# Autodesk Inventor assembly: cellSTORM_v5_microsocpe_alliedvision
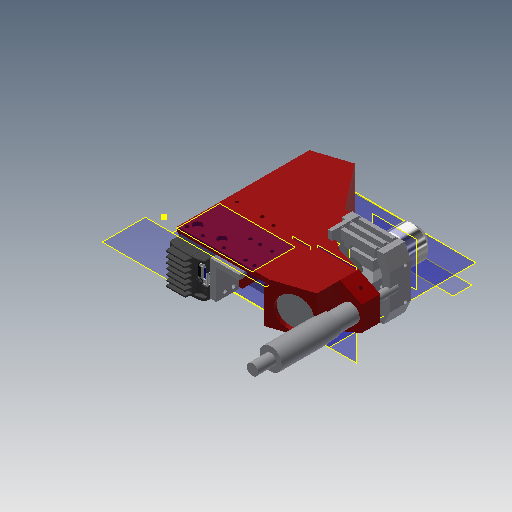
[picture p0: Inventor's stored thumbnail of the model, 512x512]
Saved by Autodesk Inventor 2019.4 (Build 234330000, 330)
## iProperties
Created: 2020-04-25
Part Number: cellSTORM_v5_microsocpe_alliedvision
Document SubType Name: Assembly
Designer: diederichbenedict
Author: diederichbenedict
## Documents named in this file (9)
- C:\Users\diederichbenedict\Dropbox\Dokumente\Promotion\PROJECTS\STORMoChip\GITHUB\CAD\Nanoscopy-on-the-cheap\Workspace\cellSTORM_v5_microsocpe_alliedvision.iam
- C:\Users\diederichbenedict\Dropbox\Dokumente\Promotion\PROJECTS\STORMoChip\GITHUB\CAD\Nanoscopy-on-the-cheap\Workspace\10_Filteslide_25mm.ipt
- C:\Users\diederichbenedict\Dropbox\Dokumente\Promotion\PROJECTS\STORMoChip\GITHUB\CAD\Nanoscopy-on-the-cheap\Workspace\cellSTORM_lightpath.ipt
- C:\Users\diederichbenedict\Dropbox\Dokumente\Promotion\PROJECTS\STORMoChip\GITHUB\CAD\Nanoscopy-on-the-cheap\Workspace\PF10-03-P01-Step.ipt
- C:\Users\diederichbenedict\Dropbox\Dokumente\Promotion\PROJECTS\STORMoChip\GITHUB\CAD\Nanoscopy-on-the-cheap\Workspace\cellSTORM_v5_opticalstage.ipt
- C:\Users\diederichbenedict\Dropbox\Dokumente\Promotion\PROJECTS\STORMoChip\GITHUB\CAD\Nanoscopy-on-the-cheap\Workspace\00_Micrometer.ipt
- C:\Users\diederichbenedict\Dropbox\Dokumente\Promotion\PROJECTS\STORMoChip\GITHUB\CAD\Nanoscopy-on-the-cheap\Workspace\Assembly_Z_stage.iam
- C:\Users\diederichbenedict\Dropbox\Dokumente\Promotion\PROJECTS\STORMoChip\GITHUB\CAD\Nanoscopy-on-the-cheap\Workspace\00_Alvium_Step_USB90_S-Mount_ClosedHousing_2019-Mar-28.ipt
- C:\Users\diederichbenedict\Dropbox\Dokumente\Promotion\PROJECTS\STORMoChip\GITHUB\CAD\Nanoscopy-on-the-cheap\Workspace\cellSTORM_alviumadapter.ipt
## Components (9 placed, 8 different names)
1. 10_Filteslide_25mm:1
2. PF10-03-P01-Step:1
3. PF10-03-P01-Step:2
4. Assembly_Z_stage:1 [sub-assembly] — Insert:7
5. cellSTORM_v5_opticalstage:1 — Insert:6, Insert:7, Insert:8, Flush:1, Flush:2, Angle:1
6. cellSTORM_lightpath:1
7. 00_Micrometer:1 — Insert:6
8. 00_Alvium_Step_USB90_S-Mount_ClosedHousing_2019-Mar-28:1 — Insert:8, Angle:1
9. cellSTORM_alviumadapter:1 — Flush:1, Flush:2
## Relationships (9: Insert 6, Flush 2, Angle 1)
- [Insert]: PF10-03-P01-Step:1 ↔ cellSTORM_lightpath:1
- [Insert]: PF10-03-P01-Step:2 ↔ cellSTORM_lightpath:1
- [Insert] (40 mm): 10_Filteslide_25mm:1 ↔ cellSTORM_lightpath:1
- Insert:6: cellSTORM_v5_opticalstage:1 ↔ 00_Micrometer:1
- Insert:7: Assembly_Z_stage:1 ↔ cellSTORM_v5_opticalstage:1
- Insert:8 (1 mm): cellSTORM_v5_opticalstage:1 ↔ 00_Alvium_Step_USB90_S-Mount_ClosedHousing_2019-Mar-28:1
- Flush:1: cellSTORM_v5_opticalstage:1 ↔ cellSTORM_alviumadapter:1
- Flush:2: cellSTORM_v5_opticalstage:1 ↔ cellSTORM_alviumadapter:1
- Angle:1 (90 deg): cellSTORM_v5_opticalstage:1 ↔ 00_Alvium_Step_USB90_S-Mount_ClosedHousing_2019-Mar-28:1
